# Autodesk Inventor assembly: XMotor
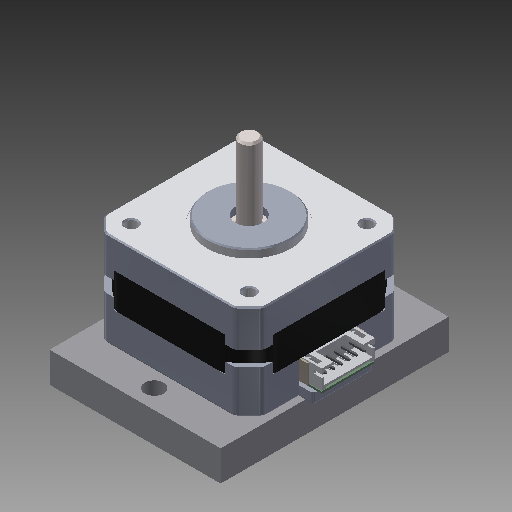
[picture p0: Inventor's stored thumbnail of the model, 512x512]
Saved by Autodesk Inventor 2019 (Build 230136000, 136)
## iProperties
Created: 2019-08-19
Part Number: XMotor
Document SubType Name: Assembly
Designer: Bruno
Mass: 55.9402 g
Surface Area: 273.893 cm^2
Volume: 55.9402 cm^3
Density: 1 g/cm^3
Author: Bruno
## Documents named in this file (3)
- C:\Users\Bruno\Stuff\Ajedrez2\XMotor.iam
- C:\Users\Bruno\Stuff\Ajedrez2\17HS10-0704S.ipt
- C:\Users\Bruno\Stuff\Ajedrez2\XMotorMount.ipt
## Components (2 placed, 2 different names)
1. 17HS10-0704S:1 — Rigid:1
2. XMotorMount:1 — Rigid:1
## Relationships (1: WeldJoint 1)
- Rigid:1 [WeldJoint]: 17HS10-0704S:1 ↔ XMotorMount:1
